# Autodesk Inventor assembly: TurretAssembly
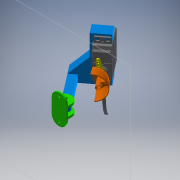
[picture p0: Inventor's stored thumbnail of the model, 180x180]
Saved by Autodesk Inventor 2016 (Build 200138000, 138)
## iProperties
Created: 2016-04-17
Part Number: TurretAssembly
Document SubType Name: Assembly
Designer: amenoni
Author: amenoni
## Documents named in this file (6)
- Z:\Desarrollo\WetMaths\wetMaths-Arduino\wetMaths\HwDesigns\TurretAssembly.iam
- Z:\Desarrollo\WetMaths\wetMaths-Arduino\wetMaths\HwDesigns\turretSupport.ipt
- Z:\Desarrollo\WetMaths\wetMaths-Arduino\wetMaths\HwDesigns\TurretServoSupport.ipt
- Z:\Desarrollo\WetMaths\wetMaths-Arduino\wetMaths\HwDesigns\Futaba S3004.ipt
- Z:\Desarrollo\WetMaths\wetMaths-Arduino\wetMaths\HwDesigns\CanNozzle.ipt
- Z:\Desarrollo\WetMaths\wetMaths-Arduino\wetMaths\HwDesigns\Servo_arm_np1.ipt
## Components (5 placed, 5 different names)
1. turretSupport:1 — Mate:1, Mate:2
2. TurretServoSupport:1 — Mate:1, Mate:2, Mate:3, Mate:4, Mate:5
3. Futaba S3004:1 — Mate:3, Mate:4, Mate:5, Mate:6, Mate:7
4. CanNozzle:1 — Mate:8, Mate:9, Mate:10
5. Servo_arm_np1:1 — Mate:6, Mate:7, Mate:8, Mate:9, Mate:10
## Relationships (10: Mate 10)
- Mate:1: turretSupport:1 ↔ TurretServoSupport:1
- Mate:2: turretSupport:1 ↔ TurretServoSupport:1
- Mate:3: TurretServoSupport:1 ↔ Futaba S3004:1
- Mate:4: TurretServoSupport:1 ↔ Futaba S3004:1
- Mate:5: TurretServoSupport:1 ↔ Futaba S3004:1
- Mate:6: Futaba S3004:1 ↔ Servo_arm_np1:1
- Mate:7: Futaba S3004:1 ↔ Servo_arm_np1:1
- Mate:8: CanNozzle:1 ↔ Servo_arm_np1:1
- Mate:9: CanNozzle:1 ↔ Servo_arm_np1:1
- Mate:10: CanNozzle:1 ↔ Servo_arm_np1:1
